# Autodesk Inventor assembly: robot
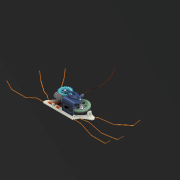
[picture p0: Inventor's stored thumbnail of the model, 180x180]
Saved by Autodesk Inventor 2020 (Build 240168000, 168)
## iProperties
Created: 2020-07-14
Part Number: robot
Document SubType Name: Assembly
Designer: alons
Author: alons
## Documents named in this file (22)
- C:\Users\alons\OneDrive\Documents\GitHub\Water-Strider-Robot\Striderbot\robot.iam
- C:\Users\alons\OneDrive\Documents\GitHub\Water-Strider-Robot\Striderbot\spur_gears_mesh_2\Design Accelerator\Spur Gear13.ipt
- C:\Users\alons\OneDrive\Documents\GitHub\Water-Strider-Robot\Striderbot\spur_gears_mesh_2\Design Accelerator\Spur Gear23.ipt
- C:\Users\alons\OneDrive\Documents\GitHub\Water-Strider-Robot\Striderbot\spur_gears_mesh_3\Design Accelerator\Spur Gear11.ipt
- C:\Users\alons\OneDrive\Documents\GitHub\Water-Strider-Robot\Striderbot\spur_gears_mesh_3\Design Accelerator\Spur Gear21.ipt
- C:\Users\alons\OneDrive\Documents\GitHub\Water-Strider-Robot\Striderbot\worm_gear_mesh_1\Design Accelerator\Worm Gear14.ipt
- C:\Users\alons\OneDrive\Documents\GitHub\Water-Strider-Robot\Striderbot\Crank_Rocker\Link_1.ipt
- C:\Users\alons\OneDrive\Documents\GitHub\Water-Strider-Robot\Striderbot\Crank_Rocker\Link_2.ipt
- C:\Users\alons\OneDrive\Documents\GitHub\Water-Strider-Robot\Striderbot\Crank_Rocker\Link_3.ipt
- C:\Users\alons\OneDrive\Documents\GitHub\Water-Strider-Robot\Striderbot\worm_gear_mesh_1\Design Accelerator\Worm14.ipt
- C:\Users\alons\OneDrive\Documents\GitHub\Water-Strider-Robot\Striderbot\Machine_Frame\top_frame.ipt
- C:\Users\alons\OneDrive\Documents\GitHub\Water-Strider-Robot\Striderbot\Machine_Frame\bottom_frame.ipt
- C:\Users\alons\OneDrive\Documents\GitHub\Water-Strider-Robot\Striderbot\Machine_Frame\bottom_frame_2.ipt
- C:\Users\alons\OneDrive\Documents\GitHub\Water-Strider-Robot\Striderbot\shafts\Shaft1.ipt
- C:\Users\alons\OneDrive\Documents\GitHub\Water-Strider-Robot\Striderbot\shafts\Shaft2.ipt
- C:\Users\alons\OneDrive\Documents\GitHub\Water-Strider-Robot\Striderbot\shafts\Shaft5.ipt
- C:\Users\alons\OneDrive\Documents\GitHub\Water-Strider-Robot\Striderbot\shafts\Shaft3.ipt
- C:\Users\alons\OneDrive\Documents\GitHub\Water-Strider-Robot\Striderbot\shafts\Shaft4.ipt
- C:\Users\alons\OneDrive\Documents\GitHub\Water-Strider-Robot\Striderbot\Machine_Frame\leg.ipt
- C:\Users\alons\OneDrive\Documents\GitHub\Water-Strider-Robot\Striderbot\Shaft1.ipt
- C:\Users\alons\OneDrive\Documents\GitHub\Water-Strider-Robot\Striderbot\Shaft2.ipt
- C:\Users\alons\OneDrive\Documents\GitHub\Water-Strider-Robot\Striderbot\Shaft3.ipt
## Components (29 placed, 14 different names)
1. Spur Gear1:1 — Flush:1, Mate:3, Rotation:1, Mate:10, Mate:11, Mate:34, Mate:43, Mate:75, Mate:78
2. Spur Gear2:1 — Flush:1, Mate:3, Rotation:1, Flush:2, Mate:6, Mate:39, Mate:56, Mate:76
3. Spur Gear1:2 — Flush:2, Mate:6, Flush:3, Mate:7, Rotation:3, Mate:19, Mate:35
4. Spur Gear2:2 — Flush:3, Mate:7, Rotation:3, Mate:12, Mate:13, Mate:14, Mate:40, Mate:73, Mate:77, Mate:79, Tangent:1, Mate:84, Mate:85
5. Worm Gear:1 — Mate:10, Mate:11, Rotation:4, Mate:32, Mate:42
6. Link_1:1 — Mate:12, Mate:13, Mate:14, Mate:15, Mate:16
7. Link_2:1 — Mate:15, Mate:16, Mate:17, Mate:18, Mate:72, Flush:10, Flush:11, Mate:86
8. Link_3:1 — Mate:17, Mate:18, Mate:19, Mate:44, Mate:68, Angle:7, Mate:69, Mate:87, Flush:13
9. Worm:1 — Rotation:4, Mate:33, Flush:8, Mate:53, Mate:80, Mate:82
10. top_frame:1 — Mate:25, Mate:26, Mate:32, Mate:33, Mate:34, Mate:35, Flush:8, Mate:39, Mate:40, Mate:42, Mate:45, Mate:82, Mate:84
11. bottom_frame:1 — Mate:25, Mate:26, Mate:41, Mate:46, Mate:47, Flush:9, Mate:50, Mate:51, Mate:58, Angle:1, Mate:59, Mate:60, Angle:2, Mate:61, Mate:62, Mate:63, Angle:3, Angle:4, Mate:64, Mate:65, Mate:66, Mate:67, Angle:5, Angle:6, Mate:70, Mate:71, Flush:12, Mate:83
12. bottom_frame_2:1 — Mate:43, Mate:44, Mate:45
13. Driving_Shaft — Mate:77, Mate:79
14. Frame_Shaft — Mate:50, Mate:51
15. Shaft:2 — Mate:75, Mate:78
16. Shaft:3 — Mate:56, Mate:76
17. Shaft:4 — Mate:53, Mate:80
18. leg:1 — Mate:58, Angle:1, Mate:59
19. leg:2 — Mate:60, Angle:2, Mate:61
20. leg:3 — Mate:62, Angle:4, Mate:64
21. leg:4 — Mate:63, Angle:3, Mate:65
22. leg:5 — Mate:67, Angle:5, Mate:71
23. leg:6 — Mate:66, Angle:6, Mate:70
24. leg:7 — Mate:68, Angle:7, Mate:69
25. Shaft:1 — Mate:72, Flush:10
26. Shaft:1 — Mate:73, Flush:11
27. Shaft:6 — Tangent:1, Flush:12, Mate:83
28. Shaft:7 — Mate:85, Mate:86
29. Shaft:8 — Mate:87, Flush:13
## Relationships (80: Mate 60, Flush 9, Angle 7, RelateRotation 3, Tangent 1)
- Flush:1: Spur Gear1:1 ↔ Spur Gear2:1
- Mate:3 (6.3 mm): Spur Gear1:1 ↔ Spur Gear2:1
- Rotation:1 [RelateRotation] (0.7812 ul): Spur Gear1:1 ↔ Spur Gear2:1
- Flush:2: Spur Gear2:1 ↔ Spur Gear1:2
- Mate:6: Spur Gear2:1 ↔ Spur Gear1:2
- Flush:3: Spur Gear1:2 ↔ Spur Gear2:2
- Mate:7 (8.45 mm): Spur Gear1:2 ↔ Spur Gear2:2
- Rotation:3 [RelateRotation] (0.789 ul): Spur Gear1:2 ↔ Spur Gear2:2
- Mate:10: Spur Gear1:1 ↔ Worm Gear:1
- Mate:11: Spur Gear1:1 ↔ Worm Gear:1
- Mate:12: Spur Gear2:2 ↔ Link_1:1
- Mate:13: Spur Gear2:2 ↔ Link_1:1
- Mate:14 (1.3 mm): Spur Gear2:2 ↔ Link_1:1
- Mate:15: Link_1:1 ↔ Link_2:1
- Mate:16: Link_1:1 ↔ Link_2:1
- Mate:17: Link_2:1 ↔ Link_3:1
- Mate:18: Link_2:1 ↔ Link_3:1
- Mate:19: Spur Gear1:2 ↔ Link_3:1
- Rotation:4 [RelateRotation] (0.0455 ul): Worm Gear:1 ↔ Worm:1
- Mate:25: top_frame:1 ↔ bottom_frame:1
- Mate:26: top_frame:1 ↔ bottom_frame:1
- Mate:32: Worm Gear:1 ↔ top_frame:1
- Mate:33: Worm:1 ↔ top_frame:1
- Mate:34 (-2 mm): Spur Gear1:1 ↔ top_frame:1
- Mate:35 (-4.2 mm): Spur Gear1:2 ↔ top_frame:1
- Flush:8 (13.55 mm): Worm:1 ↔ top_frame:1
- Mate:39 (-6.8 mm): Spur Gear2:1 ↔ top_frame:1
- Mate:40 (-6.8 mm): Spur Gear2:2 ↔ top_frame:1
- Mate:41: bottom_frame:1
- Mate:42: Worm Gear:1 ↔ top_frame:1
- Mate:43: Spur Gear1:1 ↔ bottom_frame_2:1
- Mate:44: Link_3:1 ↔ bottom_frame_2:1
- Mate:45: top_frame:1 ↔ bottom_frame_2:1
- Mate:46: bottom_frame:1
- Mate:47: bottom_frame:1
- Flush:9: bottom_frame:1
- Mate:50: bottom_frame:1 ↔ Frame_Shaft
- Mate:51: bottom_frame:1 ↔ Frame_Shaft
- Mate:53: Worm:1 ↔ Shaft:4
- Mate:56: Spur Gear2:1 ↔ Shaft:3
- Mate:58: bottom_frame:1 ↔ leg:1
- Angle:1 (90 deg): bottom_frame:1 ↔ leg:1
- Mate:59: bottom_frame:1 ↔ leg:1
- Mate:60: bottom_frame:1 ↔ leg:2
- Angle:2 (270 deg): bottom_frame:1 ↔ leg:2
- Mate:61: bottom_frame:1 ↔ leg:2
- Mate:62: bottom_frame:1 ↔ leg:3
- Mate:63: bottom_frame:1 ↔ leg:4
- Angle:3 (270 deg): bottom_frame:1 ↔ leg:4
- Angle:4 (90 deg): bottom_frame:1 ↔ leg:3
- Mate:64: bottom_frame:1 ↔ leg:3
- Mate:65: bottom_frame:1 ↔ leg:4
- Mate:66: bottom_frame:1 ↔ leg:6
- Mate:67: bottom_frame:1 ↔ leg:5
- Angle:5 (90 deg): bottom_frame:1 ↔ leg:5
- Angle:6 (270 deg): bottom_frame:1 ↔ leg:6
- Mate:68: Link_3:1 ↔ leg:7
- Angle:7 (270 deg): Link_3:1 ↔ leg:7
- Mate:69: Link_3:1 ↔ leg:7
- Mate:70: bottom_frame:1 ↔ leg:6
- Mate:71: bottom_frame:1 ↔ leg:5
- Mate:72: Link_2:1 ↔ Shaft:1
- Flush:10: Link_2:1 ↔ Shaft:1
- Mate:73: Spur Gear2:2 ↔ Shaft:1
- Flush:11: Link_2:1 ↔ Shaft:1
- Mate:75: Spur Gear1:1 ↔ Shaft:2
- Mate:76: Spur Gear2:1 ↔ Shaft:3
- Mate:77: Spur Gear2:2 ↔ Driving_Shaft
- Mate:78: Spur Gear1:1 ↔ Shaft:2
- Mate:79: Spur Gear2:2 ↔ Driving_Shaft
- Mate:80: Worm:1 ↔ Shaft:4
- Mate:82: Worm:1 ↔ top_frame:1
- Tangent:1: Spur Gear2:2 ↔ Shaft:6
- Flush:12: bottom_frame:1 ↔ Shaft:6
- Mate:83: bottom_frame:1 ↔ Shaft:6
- Mate:84: Spur Gear2:2 ↔ top_frame:1
- Mate:85: Spur Gear2:2 ↔ Shaft:7
- Mate:86: Link_2:1 ↔ Shaft:7
- Mate:87: Link_3:1 ↔ Shaft:8
- Flush:13: Link_3:1 ↔ Shaft:8
